# Autodesk Inventor assembly: Base
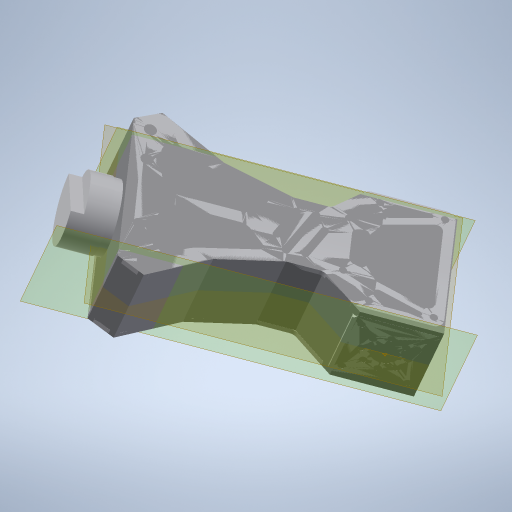
[picture p0: Inventor's stored thumbnail of the model, 512x512]
Saved by Autodesk Inventor 2023 (Build 270158000, 158)
## iProperties
Created: 2020-03-24
Part Number: Base
Document SubType Name: Assembly
Designer: valer
Mass: 1090.49 g
Surface Area: 1238.82 cm^2
Volume: 758.006 cm^3
Density: 1.43863 g/cm^3
Author: valer
## Documents named in this file (9)
- C:\Users\LattePanda\Desktop\str1ker\cad\ArmBase.iam
- C:\Users\LattePanda\Desktop\str1ker\cad\external\ShoulderActuator\ShoulderActuator.ipt
- C:\Users\LattePanda\Desktop\str1ker\cad\external\ShoulderMiterGear.ipt
- C:\Users\LattePanda\Desktop\str1ker\cad\external\ShoulderActuator\ShoulderActuatorShaft.ipt
- C:\Users\LattePanda\Desktop\str1ker\cad\external\ShoulderMotorMount.ipt
- C:\Users\LattePanda\Desktop\str1ker\cad\external\PatternSpacer.ipt
- C:\Users\LattePanda\Desktop\str1ker\cad\ShoulderBracket.ipt
- C:\Users\LattePanda\Desktop\str1ker\cad\external\Potentiometer\Potentiometer.iam
- C:\Users\LattePanda\Desktop\str1ker\cad\BaseBoundingBox.ipt
## Components (11 placed, 8 different names)
1. ShoulderServo:1 — Mate:301, Mate:367, Mate:368
2. ShoulderMiterGear:1 — Mate:303, Mate:369
3. ShoulderServoShaft:1 — Mate:301, Mate:303, Mate:316, Mate:367
4. ShoulderMotorMount:1 — Mate:316, Mate:326, Mate:365, Mate:366, Mate:368, Mate:369
5. ShoulderMotorMount:2 — Mate:321, Mate:323, Mate:324, Mate:325, Mate:328, Mate:364, Mate:370, Mate:371
6. PatternSpacer:1 — Mate:321, Mate:370, Mate:371, Mate:375, Mate:376
7. ShoulderBracket:1 — Mate:323, Mate:324, Mate:325, Mate:365, Mate:366, Mate:373, Angle:3, Flush:1
8. ShoulderBracket:2 — Mate:326, Mate:328, Mate:359, Mate:360, Mate:361, Mate:364, Angle:4
9. ShoulderMotorMount:3 — Mate:359, Mate:360, Mate:361, Mate:372, Mate:373, Mate:374, Angle:2, Mate:377
10. Potentiometer:1 [sub-assembly] — Mate:372, Mate:374, Angle:2
11. BaseBoundingBox:1 — Mate:375, Angle:4, Flush:1
## Relationships (30: Mate 26, Angle 3, Flush 1)
- Mate:301: ShoulderServo:1 ↔ ShoulderServoShaft:1
- Mate:303: ShoulderMiterGear:1 ↔ ShoulderServoShaft:1
- Mate:316: ShoulderServoShaft:1 ↔ ShoulderMotorMount:1
- Mate:321: ShoulderMotorMount:2 ↔ PatternSpacer:1
- Mate:323: ShoulderMotorMount:2 ↔ ShoulderBracket:1
- Mate:324: ShoulderMotorMount:2 ↔ ShoulderBracket:1
- Mate:325: ShoulderMotorMount:2 ↔ ShoulderBracket:1
- Mate:326: ShoulderMotorMount:1 ↔ ShoulderBracket:2
- Mate:328: ShoulderMotorMount:2 ↔ ShoulderBracket:2
- Mate:359: ShoulderBracket:2 ↔ ShoulderMotorMount:3
- Mate:360: ShoulderBracket:2 ↔ ShoulderMotorMount:3
- Mate:361: ShoulderBracket:2 ↔ ShoulderMotorMount:3
- Mate:364: ShoulderMotorMount:2 ↔ ShoulderBracket:2
- Mate:365: ShoulderMotorMount:1 ↔ ShoulderBracket:1
- Mate:366: ShoulderMotorMount:1 ↔ ShoulderBracket:1
- Mate:367 (-4 mm): ShoulderServo:1 ↔ ShoulderServoShaft:1
- Mate:368: ShoulderServo:1 ↔ ShoulderMotorMount:1
- Mate:369 (1 mm): ShoulderMiterGear:1 ↔ ShoulderMotorMount:1
- Mate:370: ShoulderMotorMount:2 ↔ PatternSpacer:1
- Mate:371: ShoulderMotorMount:2 ↔ PatternSpacer:1
- Mate:372: ShoulderMotorMount:3 ↔ Potentiometer:1
- Mate:373: ShoulderBracket:1 ↔ ShoulderMotorMount:3
- Mate:374: ShoulderMotorMount:3 ↔ Potentiometer:1
- Angle:2 (0 deg): ShoulderMotorMount:3 ↔ Potentiometer:1
- Angle:3 (0 deg): ShoulderBracket:1
- Mate:375: PatternSpacer:1 ↔ BaseBoundingBox:1
- Angle:4 (0 deg): ShoulderBracket:2 ↔ BaseBoundingBox:1
- Mate:376: PatternSpacer:1
- Mate:377: ShoulderMotorMount:3
- Flush:1: ShoulderBracket:1 ↔ BaseBoundingBox:1
